# Autodesk Inventor assembly: LongTop
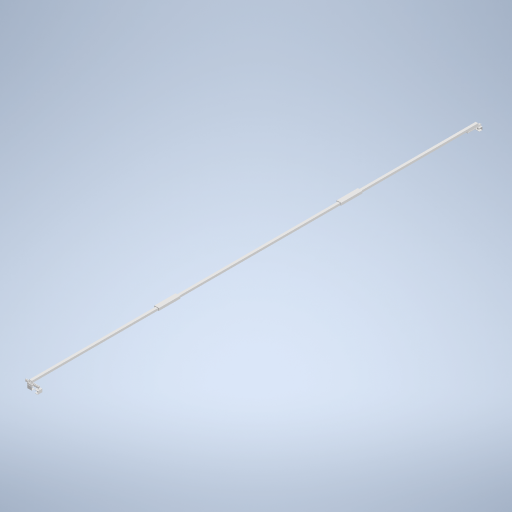
[picture p0: Inventor's stored thumbnail of the model, 512x512]
Saved by Autodesk Inventor 2023 (Build 270158030, 158C)
## iProperties
Created: 2022-06-29
Part Number: LongTop
Document SubType Name: Assembly
Designer: jeremyy
Author: jeremyy
## Documents named in this file (8)
- \\andrew.ad.cmu.edu\users\users1\jeremyy\Documents\Inventor\CMU Bridge\New folder\LongTop.iam
- \\andrew.ad.cmu.edu\users\users1\jeremyy\Documents\Inventor\CMU Bridge\New folder\LongStrut84Sec1.ipt
- \\andrew.ad.cmu.edu\users\users1\jeremyy\Documents\Inventor\CMU Bridge\New folder\LongStrut90Sec3.ipt
- \\andrew.ad.cmu.edu\users\users1\jeremyy\Documents\Inventor\CMU Bridge\New folder\LongStrut120Sec2.ipt
- \\andrew.ad.cmu.edu\users\users1\jeremyy\Documents\Inventor\CMU Bridge\New folder\LongC3x6Top14in.ipt
- \\andrew.ad.cmu.edu\users\users1\jeremyy\Documents\Inventor\CMU Bridge\New folder\VertX3in.ipt
- \\andrew.ad.cmu.edu\users\users1\jeremyy\Documents\Inventor\CMU Bridge\New folder\Gear.iam
- \\andrew.ad.cmu.edu\users\users1\jeremyy\Documents\Inventor\CMU Bridge\New folder\VertX9in.ipt
## Components (11 placed, 7 different names)
1. LongStrut84Sec1:1 — Mate:1, Flush:1, Mate:2, Mate:3, Mate:19, Flush:9, Flush:10
2. LongStrut90Sec3:1 — Mate:8, Mate:9, Mate:10, Mate:11, Flush:3, Flush:4, Mate:16, Flush:6
3. LongStrut120Sec2:1 — Mate:3, Mate:4, Mate:5, Flush:2, Mate:6, Mate:7, Mate:8
4. LongC3x6Top14in:1 — Flush:2, Mate:6, Mate:7, Mate:9, Mate:10
5. LongC3x6Top14in:2 — Mate:1, Flush:1, Mate:2, Mate:4, Mate:5
6. VertX3in:1 — Mate:11, Flush:3, Flush:4, Mate:15, Flush:5, Mate:17
7. Gear:1 [sub-assembly] — Mate:15, Flush:5
8. Gear:2 [sub-assembly] — Mate:18, Flush:7, Flush:8
9. VertX9in:1 — Mate:16, Flush:6, Mate:17, Mate:18, Flush:7, Flush:8
10. VertX9in:2 — Mate:19, Flush:9, Flush:10, Mate:20, Flush:11
11. Gear:3 [sub-assembly] — Mate:20, Flush:11
## Relationships (28: Mate 17, Flush 11)
- Mate:1: LongStrut84Sec1:1 ↔ LongC3x6Top14in:2
- Flush:1 (177.8 mm): LongStrut84Sec1:1 ↔ LongC3x6Top14in:2
- Mate:2 (8.636 mm): LongStrut84Sec1:1 ↔ LongC3x6Top14in:2
- Mate:3: LongStrut84Sec1:1 ↔ LongStrut120Sec2:1
- Mate:4 (8.636 mm): LongStrut120Sec2:1 ↔ LongC3x6Top14in:2
- Mate:5: LongStrut120Sec2:1 ↔ LongC3x6Top14in:2
- Flush:2 (-177.8 mm): LongStrut120Sec2:1 ↔ LongC3x6Top14in:1
- Mate:6: LongStrut120Sec2:1 ↔ LongC3x6Top14in:1
- Mate:7 (8.636 mm): LongStrut120Sec2:1 ↔ LongC3x6Top14in:1
- Mate:8: LongStrut90Sec3:1 ↔ LongStrut120Sec2:1
- Mate:9 (8.636 mm): LongStrut90Sec3:1 ↔ LongC3x6Top14in:1
- Mate:10: LongStrut90Sec3:1 ↔ LongC3x6Top14in:1
- Mate:11: LongStrut90Sec3:1 ↔ VertX3in:1
- Flush:3 (-38.1 mm): LongStrut90Sec3:1 ↔ VertX3in:1
- Flush:4 (12.7 mm): LongStrut90Sec3:1 ↔ VertX3in:1
- Mate:15: VertX3in:1 ↔ Gear:1
- Flush:5: VertX3in:1 ↔ Gear:1
- Mate:16: LongStrut90Sec3:1 ↔ VertX9in:1
- Flush:6 (-76.2 mm): LongStrut90Sec3:1 ↔ VertX9in:1
- Mate:17: VertX3in:1 ↔ VertX9in:1
- Mate:18: Gear:2 ↔ VertX9in:1
- Flush:7 (-25.4 mm): Gear:2 ↔ VertX9in:1
- Flush:8 (38.1 mm): Gear:2 ↔ VertX9in:1
- Mate:19: LongStrut84Sec1:1 ↔ VertX9in:2
- Flush:9: LongStrut84Sec1:1 ↔ VertX9in:2
- Flush:10 (-50.8 mm): LongStrut84Sec1:1 ↔ VertX9in:2
- Mate:20: VertX9in:2 ↔ Gear:3
- Flush:11: VertX9in:2 ↔ Gear:3
